# Autodesk Inventor assembly: robot_assembly
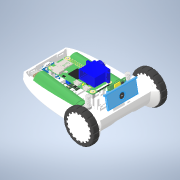
[picture p0: Inventor's stored thumbnail of the model, 180x180]
Saved by Autodesk Inventor 2022.1 (Build 261234020, 234B)
## iProperties
Created: 2021-07-07
Part Number: robot_assembly
Document SubType Name: Assembly
Designer: dwbertol
Author: dwbertol
## Documents named in this file (22)
- C:\Users\dwbertol\Desktop\robot\v2\robot_assembly.iam
- C:\Users\dwbertol\Desktop\robot\v2\base.ipt
- C:\Users\dwbertol\Desktop\robot\v2\driver.ipt
- C:\Users\dwbertol\Desktop\robot\v2\rpi.ipt
- C:\Users\dwbertol\Desktop\robot\v2\bussola.ipt
- C:\Users\dwbertol\Desktop\robot\v2\cam.ipt
- C:\Users\dwbertol\Desktop\robot\v2\front.ipt
- C:\Users\dwbertol\Desktop\robot\v2\GearMotor\Motor.iam
- C:\Users\dwbertol\Desktop\robot\v2\battery.ipt
- C:\Users\dwbertol\Desktop\robot\v2\charger.ipt
- C:\Users\dwbertol\Desktop\robot\v2\step_down.ipt
- C:\Users\dwbertol\Desktop\robot\v2\step_up.ipt
- C:\Users\dwbertol\Desktop\robot\v2\top.ipt
- C:\Users\dwbertol\Desktop\robot\v2\small_switch.ipt
- C:\Users\dwbertol\Desktop\robot\v2\wheel.ipt
- C:\Users\dwbertol\Desktop\robot\v2\tire.ipt
- C:\Users\dwbertol\Desktop\robot\v2\bolt.ipt
- C:\Users\dwbertol\Desktop\robot\v2\servo.ipt
- C:\Users\dwbertol\Desktop\robot\v2\giro.ipt
- C:\Users\dwbertol\Desktop\robot\v2\rpi_base_back.ipt
- C:\Users\dwbertol\Desktop\robot\v2\rpi_base_front.ipt
- C:\Users\dwbertol\Desktop\robot\v2\washer.ipt
## Components (29 placed, 21 different names)
1. base:1 — Angle:4, Mate:17, Mate:27, Mate:34, Mate:35, Mate:36, Mate:37, Mate:38, Mate:39, Mate:40, Mate:44, Mate:47, Mate:50, Angle:5, Mate:58, Mate:74, Flush:3, Flush:4, Mate:91, Mate:93, Mate:94, Mate:95, Mate:100, Mate:103, Mate:105, Mate:106, Mate:107, Mate:124, Mate:129, Mate:130, Mate:131, Mate:132, Mate:133, Mate:134, Mate:135, Mate:136, Mate:140, Mate:141, Mate:142, Mate:143, Mate:146, Mate:147, Mate:148, Angle:9, Mate:149, Angle:10, Mate:150, Mate:151, Angle:11, Angle:12, Mate:154, Mate:155, Mate:156, Mate:157, Mate:163, Mate:164
2. top:1 — Flush:3, Flush:4, Mate:91, Mate:111, Mate:112, Mate:144
3. cam:1 — Mate:158, Mate:159, Angle:13
4. front:1 — Mate:111, Mate:112, Mate:158, Mate:159, Angle:13
5. GearMotor:1 [sub-assembly] — Angle:4, Mate:17, Mate:27, Mate:98, Angle:7
6. GearMotor:2 [sub-assembly] — Angle:5, Mate:58, Mate:101, Angle:8, Mate:124
7. rpi:1 — Mate:160, Mate:161, Mate:162
8. battery:1 — Mate:34, Mate:36
9. battery:2 — Mate:35, Mate:37
10. charger:1 — Mate:38, Mate:39, Mate:40
11. bussola:1 — Mate:74, Mate:134, Mate:135
12. driver:1 — Mate:50, Mate:142, Mate:143
13. step_down:1 — Mate:47, Mate:132, Mate:133
14. step_up:1 — Mate:44, Mate:130, Mate:131
15. small_switch:1 — Mate:93, Mate:94, Mate:95
16. wheel:1 — Mate:97, Flush:7, Mate:101, Angle:8, Mate:102, Mate:103
17. wheel:2 — Mate:96, Flush:6, Mate:98, Angle:7, Mate:99, Mate:100
18. tire:1 — Mate:96, Flush:6, Mate:99
19. tire:2 — Mate:97, Flush:7, Mate:102
20. bolt:1 — Mate:105, Mate:129
21. bolt:3 — Mate:106, Mate:107
22. servo:1 — Mate:144
23. giro:1 — Mate:136, Mate:140, Mate:141
24. rpi_base_back:1 — Mate:146, Mate:149, Angle:10, Mate:160, Mate:161
25. rpi_base_back:2 — Mate:147, Mate:148, Angle:9, Mate:162
26. rpi_base_front:1 — Mate:150, Angle:11, Mate:163
27. rpi_base_front:2 — Mate:151, Angle:12, Mate:164
28. washer:1 — Mate:156, Mate:157
29. washer:2 — Mate:154, Mate:155
## Relationships (75: Mate 62, Angle 9, Flush 4)
- Angle:4 (0 deg): base:1 ↔ GearMotor:1
- Mate:17: base:1 ↔ GearMotor:1
- Mate:27: base:1 ↔ GearMotor:1
- Mate:34: base:1 ↔ battery:1
- Mate:35: base:1 ↔ battery:2
- Mate:36 (7 mm): base:1 ↔ battery:1
- Mate:37 (6 mm): base:1 ↔ battery:2
- Mate:38 (0.2 mm): base:1 ↔ charger:1
- Mate:39: base:1 ↔ charger:1
- Mate:40: base:1 ↔ charger:1
- Mate:44 (0.2 mm): base:1 ↔ step_up:1
- Mate:47 (0.2 mm): base:1 ↔ step_down:1
- Mate:50 (0.2 mm): base:1 ↔ driver:1
- Angle:5 (0 deg): base:1 ↔ GearMotor:2
- Mate:58: base:1 ↔ GearMotor:2
- Mate:74 (2 mm): base:1 ↔ bussola:1
- Flush:3: base:1 ↔ top:1
- Flush:4: base:1 ↔ top:1
- Mate:91 (0.2 mm): base:1 ↔ top:1
- Mate:93: base:1 ↔ small_switch:1
- Mate:94 (0.3 mm): base:1 ↔ small_switch:1
- Mate:95 (0.3 mm): base:1 ↔ small_switch:1
- Mate:96: wheel:2 ↔ tire:1
- Flush:6: wheel:2 ↔ tire:1
- Mate:97: wheel:1 ↔ tire:2
- Flush:7: wheel:1 ↔ tire:2
- Mate:98: GearMotor:1 ↔ wheel:2
- Angle:7 (0 deg): GearMotor:1 ↔ wheel:2
- Mate:99: wheel:2 ↔ tire:1
- Mate:100: base:1 ↔ wheel:2
- Mate:101: GearMotor:2 ↔ wheel:1
- Angle:8 (0 deg): GearMotor:2 ↔ wheel:1
- Mate:102: wheel:1 ↔ tire:2
- Mate:103 (0.1 mm): base:1 ↔ wheel:1
- Mate:105: base:1 ↔ bolt:1
- Mate:106: base:1 ↔ bolt:3
- Mate:107: base:1 ↔ bolt:3
- Mate:111: top:1 ↔ front:1
- Mate:112 (0.3 mm): top:1 ↔ front:1
- Mate:124: base:1 ↔ GearMotor:2
- Mate:129: base:1 ↔ bolt:1
- Mate:130: base:1 ↔ step_up:1
- Mate:131: base:1 ↔ step_up:1
- Mate:132: base:1 ↔ step_down:1
- Mate:133: base:1 ↔ step_down:1
- Mate:134: base:1 ↔ bussola:1
- Mate:135: base:1 ↔ bussola:1
- Mate:136 (0.2 mm): base:1 ↔ giro:1
- Mate:140: base:1 ↔ giro:1
- Mate:141: base:1 ↔ giro:1
- Mate:142: base:1 ↔ driver:1
- Mate:143: base:1 ↔ driver:1
- Mate:144: top:1 ↔ servo:1
- Mate:146: base:1 ↔ rpi_base_back:1
- Mate:147: base:1 ↔ rpi_base_back:2
- Mate:148: base:1 ↔ rpi_base_back:2
- Angle:9 (0 deg): base:1 ↔ rpi_base_back:2
- Mate:149: base:1 ↔ rpi_base_back:1
- Angle:10 (0 deg): base:1 ↔ rpi_base_back:1
- Mate:150: base:1 ↔ rpi_base_front:1
- Mate:151: base:1 ↔ rpi_base_front:2
- Angle:11 (0 deg): base:1 ↔ rpi_base_front:1
- Angle:12 (0 deg): base:1 ↔ rpi_base_front:2
- Mate:154: base:1 ↔ washer:2
- Mate:155: base:1 ↔ washer:2
- Mate:156: base:1 ↔ washer:1
- Mate:157: base:1 ↔ washer:1
- Mate:158: cam:1 ↔ front:1
- Mate:159: cam:1 ↔ front:1
- Angle:13 (0 deg): cam:1 ↔ front:1
- Mate:160: rpi:1 ↔ rpi_base_back:1
- Mate:161: rpi:1 ↔ rpi_base_back:1
- Mate:162: rpi:1 ↔ rpi_base_back:2
- Mate:163: base:1 ↔ rpi_base_front:1
- Mate:164: base:1 ↔ rpi_base_front:2
